# Autodesk Inventor assembly: AC254-030-OnPost
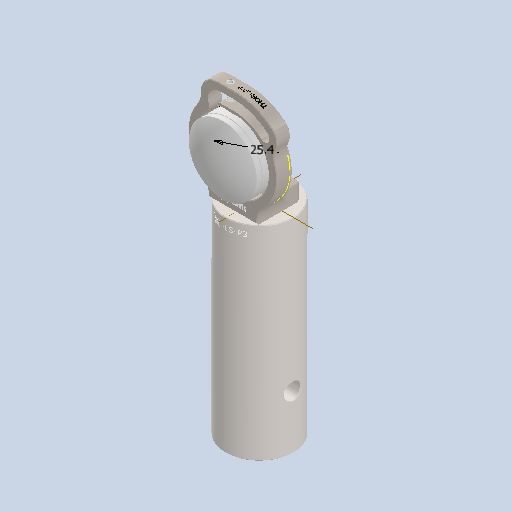
[picture p0: Inventor's stored thumbnail of the model, 512x512]
Saved by Autodesk Inventor 2025.2 (Build 292293000, 293)
## iProperties
Created: 2024-01-26
Part Number: AC254-030-OnPost
Document SubType Name: Assembly
Designer: monolithic
Author: monolithic
## Documents named in this file (3)
- C:\Users\monolithic\Documents\GitHub\CAD\Monolith\John\Altair_PowellBaseplate_SPIM_ASLM_CTASLM\Assembly\SubAssemblies\AC254-030-OnPost.iam
- C:\Users\monolithic\Documents\GitHub\CAD\Monolith\John\Altair_PowellBaseplate_SPIM_ASLM_CTASLM\Assembly\SubAssemblies\AC254-030-A-Step.ipt
- C:\Users\monolithic\Documents\GitHub\CAD\Monolith\John\Altair_PowellBaseplate_SPIM_ASLM_CTASLM\Assembly\SubAssemblies\PostLensHolder_B1S_PLS3in.iam
## Components (2 placed, 2 different names)
1. AC254-030-A-Step:1 — Insert:1
2. PostLensHolder_B1S_PLS3in:1 [sub-assembly] — Insert:1, Mate:1, Angle:1
## Relationships (3: Insert 1, Mate 1, Angle 1)
- Insert:1: AC254-030-A-Step:1 ↔ PostLensHolder_B1S_PLS3in:1
- Mate:1: PostLensHolder_B1S_PLS3in:1
- Angle:1 (0 deg): PostLensHolder_B1S_PLS3in:1
